# Autodesk Inventor assembly: inside6motorbearing
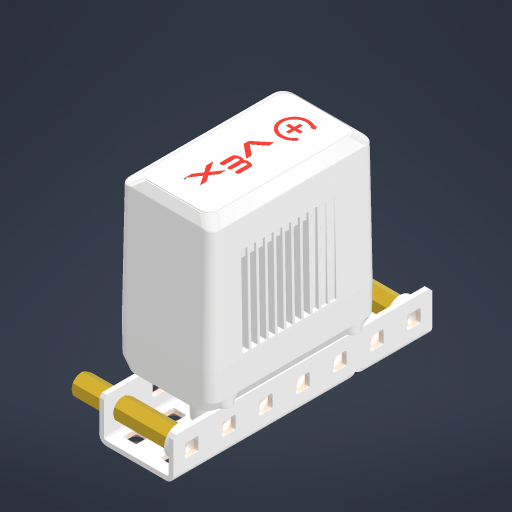
[picture p0: Inventor's stored thumbnail of the model, 512x512]
Saved by Autodesk Inventor 2023 (Build 270158000, 158)
## iProperties
Created: 2023-08-06
Part Number: inside6motorbearing
Document SubType Name: Assembly
Designer: srbel
Author: srbel
## Documents named in this file (8)
- C:\CAD\OverUnderCAD\Drive\inside6motorbearing.iam
- C:\CAD\OverUnderCAD\VEX-CAD-Inventor-1.4.0\Structure\Standoff\Standoff .50.ipt
- C:\CAD\OverUnderCAD\VEX-CAD-Inventor-1.4.0\Structure\Standoff.ipt
- C:\CAD\OverUnderCAD\VEX-CAD-Inventor-1.4.0\Structure\Standoff\Standoff .75.ipt
- C:\CAD\OverUnderCAD\VEX-CAD-Inventor-1.4.0\Motion\Spacers\Spacer Nylon .313 OD\NSpacer .313 OD x .125.ipt
- C:\CAD\OverUnderCAD\VEX-CAD-Inventor-1.4.0\Motion\Spacers\Spacer Nylon .313 OD.ipt
- C:\CAD\OverUnderCAD\VEX-CAD-Inventor-1.4.0\Structure\C Channel\Aluminum 1x2x1\Alu C 1x2x1x7.ipt
- C:\CAD\OverUnderCAD\VEX-CAD-Inventor-1.4.0\Electronics\V5 Motor.ipt
## Components (8 placed, 5 different names)
1. Standoff .50:1 — Insert:3
2. Standoff .75:2
3. NSpacer .313 OD x .125:1 — Insert:2
4. Alu C 1x2x1x7:1 — Insert:2, Insert:3, Insert:5, Insert:6, Insert:7, Insert:8
5. Standoff .75:3
6. NSpacer .313 OD x .125:2 — Insert:5
7. Standoff .50:4 — Insert:6
8. V5 Motor:1 — Insert:7, Insert:8
## Relationships (8: Insert 8)
- [Insert]: Standoff .75:2 ↔ NSpacer .313 OD x .125:1
- Insert:2: NSpacer .313 OD x .125:1 ↔ Alu C 1x2x1x7:1
- Insert:3: Standoff .50:1 ↔ Alu C 1x2x1x7:1
- [Insert]: Standoff .75:3 ↔ NSpacer .313 OD x .125:2
- Insert:5: Alu C 1x2x1x7:1 ↔ NSpacer .313 OD x .125:2
- Insert:6: Alu C 1x2x1x7:1 ↔ Standoff .50:4
- Insert:7: Alu C 1x2x1x7:1 ↔ V5 Motor:1
- Insert:8: Alu C 1x2x1x7:1 ↔ V5 Motor:1
## Named parameters: d3_d4 = 0 mm
